# Autodesk Inventor assembly: MG-Dribbler Zwischenzahnrad
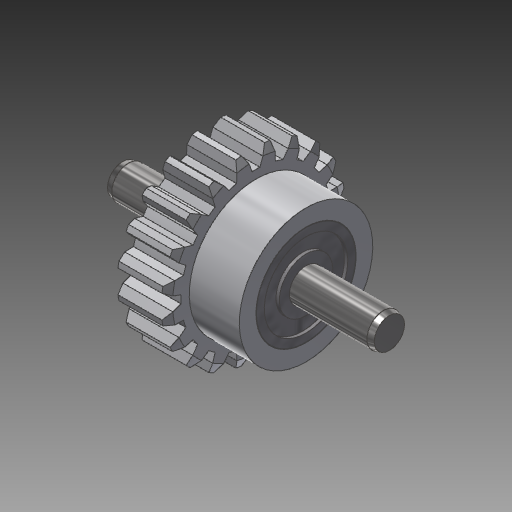
[picture p0: Inventor's stored thumbnail of the model, 512x512]
Saved by Autodesk Inventor 2019.4 (Build 234330000, 330)
## iProperties
Part Number: MG-Dribbler Zwischenzahnrad
Material: Generisch
Document SubType Name: Assembly
Designer: rYan
Mass: 1.79575 g
Surface Area: 8.35412 cm^2
Volume: 0.406946 cm^3
Density: 4.41275 g/cm^3
Author: rYan
## Documents named in this file (4)
- D:\TIGERsGIT\Hardware\mechanik\2020\Inventor\Robot\Dribbler\MG-Dribbler Zwischenzahnrad.iam
- D:\TIGERsGIT\Hardware\mechanik\2020\Inventor\Purchased Parts\Zahnrad Polyketon z20.ipt
- D:\TIGERsGIT\Hardware\mechanik\2020\Inventor\Purchased Parts\Kugellager 692-ZZ.ipt
- D:\TIGERsGIT\Hardware\mechanik\2020\Inventor\Inhaltscenter\de-DE\ISO 2338(1)\DIN EN ISO 2338 - 2 m6 x 16.ipt
## Components (4 placed, 3 different names)
1. Zahnrad Polyketon z20:1 — Fluchtend:1, Fluchtend:2, Fluchtend:3, Einfügen:1, Einfügen:2
2. Kugellager 692-ZZ:1 — Einfügen:1
3. Kugellager 692-ZZ:2 — Einfügen:2, Einfügen:3
4. DIN EN ISO 2338 2 m6 x 16:1 — Einfügen:3
## Relationships (6: Flush 3, Insert 3)
- Fluchtend:1 [Flush]: Zahnrad Polyketon z20:1
- Fluchtend:2 [Flush]: Zahnrad Polyketon z20:1
- Fluchtend:3 [Flush]: Zahnrad Polyketon z20:1
- Einfügen:1 [Insert]: Zahnrad Polyketon z20:1 ↔ Kugellager 692-ZZ:1
- Einfügen:2 [Insert]: Zahnrad Polyketon z20:1 ↔ Kugellager 692-ZZ:2
- Einfügen:3 [Insert] (-5 mm): Kugellager 692-ZZ:2 ↔ DIN EN ISO 2338 2 m6 x 16:1
